# Autodesk Inventor assembly: GE-13023
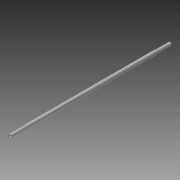
[picture p0: Inventor's stored thumbnail of the model, 180x180]
Saved by Autodesk Inventor 2013 (Build 170138000, 138)
## iProperties
Created: 2013-01-06
Part Number: GE-13023
Document SubType Name: Assembly
Designer: Phillip
Author: Phillip
## Documents named in this file (3)
- C:\Users\Moses\Documents\Inventor\2013 Team 3061 Robot\FIRST Arena 2013\Pyramid\GE-13023.iam
- C:\Users\Moses\Documents\Inventor\2013 Team 3061 Robot\FIRST Arena 2013\Pyramid\GE-13023-01.ipt
- C:\Users\Moses\Documents\Inventor\2013 Team 3061 Robot\FIRST Arena 2013\Pyramid\GE-13023-02.ipt
## Components (3 placed, 2 different names)
1. GE-13023-01:1 — Insert:1, Insert:2
2. GE-13023-02:1 — Insert:1
3. GE-13023-02:2 — Insert:2
## Relationships (2: Insert 2)
- Insert:1 (-146.05 mm): GE-13023-01:1 ↔ GE-13023-02:1
- Insert:2 (-146.05 mm): GE-13023-01:1 ↔ GE-13023-02:2
